# Autodesk Inventor assembly: HopperAssembly_v3
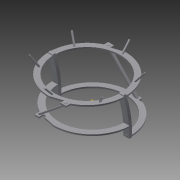
[picture p0: Inventor's stored thumbnail of the model, 180x180]
Saved by Autodesk Inventor 2013 (Build 170138000, 138)
## iProperties
Created: 2013-01-17
Part Number: HopperAssembly_v3
Document SubType Name: Assembly
Designer: twsass
Author: twsass
## Documents named in this file (8)
- E:\Robotics\Hopper\HopperAssembly_v3.iam
- E:\Robotics\Hopper\TopHoopSection_v4.ipt
- E:\Robotics\Hopper\HopperFrontSupport_v2.ipt
- E:\Robotics\Hopper\BottomHoop_v1.ipt
- E:\Robotics\Hopper\MiddleHoop.ipt
- E:\Robotics\Hopper\1Piecelongsupport_v1.ipt
- E:\Robotics\Hopper\1Pieceshortsupport_v1.ipt
- E:\Robotics\Hopper\Funneling_v1.ipt
## Components (14 placed, 7 different names)
1. TopHoopSection_v4:1 — Mate:113, Mate:114, Mate:115, Mate:131, Mate:132, Mate:133, Mate:134, Mate:135, Mate:136, Mate:137, Mate:138, Mate:139
2. HopperFrontSupport_v2:2 — Mate:78, Mate:79, Mate:80, Mate:107, Mate:108, Mate:109, Mate:116, Mate:117, Mate:118
3. TopHoopSection_v4:2 — Mate:116, Mate:117, Mate:118, Mate:122, Mate:123, Mate:124, Mate:125, Mate:126, Mate:127, Mate:128, Mate:129, Mate:130
4. BottomHoop_v1:1 — Mate:64, Mate:65, Mate:66, Mate:78, Mate:79, Mate:80, Mate:87, Mate:119, Mate:120, Mate:121
5. MiddleHoop:1 — Mate:107, Mate:108, Mate:109, Mate:110, Mate:111, Mate:112
6. HopperFrontSupport_v2:3 — Mate:64, Mate:65, Mate:66, Mate:113, Mate:114, Mate:115
7. 1Piecelongsupport_v1:1 — Mate:87, Mate:119, Mate:120, Mate:121
8. 1Pieceshortsupport_v1:1 — Mate:110, Mate:111, Mate:112
9. Funneling_v1:1 — Mate:134, Mate:135, Mate:136
10. Funneling_v1:2 — Mate:122, Mate:123, Mate:124
11. Funneling_v1:3 — Mate:131, Mate:132, Mate:133
12. Funneling_v1:4 — Mate:125, Mate:126, Mate:127
13. Funneling_v1:5 — Mate:137, Mate:138, Mate:139
14. Funneling_v1:6 — Mate:128, Mate:129, Mate:130
## Relationships (40: Mate 40)
- Mate:64: BottomHoop_v1:1 ↔ HopperFrontSupport_v2:3
- Mate:65: BottomHoop_v1:1 ↔ HopperFrontSupport_v2:3
- Mate:66: BottomHoop_v1:1 ↔ HopperFrontSupport_v2:3
- Mate:78: HopperFrontSupport_v2:2 ↔ BottomHoop_v1:1
- Mate:79: HopperFrontSupport_v2:2 ↔ BottomHoop_v1:1
- Mate:80: HopperFrontSupport_v2:2 ↔ BottomHoop_v1:1
- Mate:87: BottomHoop_v1:1 ↔ 1Piecelongsupport_v1:1
- Mate:107: HopperFrontSupport_v2:2 ↔ MiddleHoop:1
- Mate:108: HopperFrontSupport_v2:2 ↔ MiddleHoop:1
- Mate:109: HopperFrontSupport_v2:2 ↔ MiddleHoop:1
- Mate:110: MiddleHoop:1 ↔ 1Pieceshortsupport_v1:1
- Mate:111: MiddleHoop:1 ↔ 1Pieceshortsupport_v1:1
- Mate:112: MiddleHoop:1 ↔ 1Pieceshortsupport_v1:1
- Mate:113: TopHoopSection_v4:1 ↔ HopperFrontSupport_v2:3
- Mate:114: TopHoopSection_v4:1 ↔ HopperFrontSupport_v2:3
- Mate:115: TopHoopSection_v4:1 ↔ HopperFrontSupport_v2:3
- Mate:116: HopperFrontSupport_v2:2 ↔ TopHoopSection_v4:2
- Mate:117: HopperFrontSupport_v2:2 ↔ TopHoopSection_v4:2
- Mate:118: HopperFrontSupport_v2:2 ↔ TopHoopSection_v4:2
- Mate:119: BottomHoop_v1:1 ↔ 1Piecelongsupport_v1:1
- Mate:120: BottomHoop_v1:1 ↔ 1Piecelongsupport_v1:1
- Mate:121: BottomHoop_v1:1 ↔ 1Piecelongsupport_v1:1
- Mate:122: TopHoopSection_v4:2 ↔ Funneling_v1:2
- Mate:123: TopHoopSection_v4:2 ↔ Funneling_v1:2
- Mate:124: TopHoopSection_v4:2 ↔ Funneling_v1:2
- Mate:125: TopHoopSection_v4:2 ↔ Funneling_v1:4
- Mate:126: TopHoopSection_v4:2 ↔ Funneling_v1:4
- Mate:127: TopHoopSection_v4:2 ↔ Funneling_v1:4
- Mate:128: TopHoopSection_v4:2 ↔ Funneling_v1:6
- Mate:129: TopHoopSection_v4:2 ↔ Funneling_v1:6
- Mate:130: TopHoopSection_v4:2 ↔ Funneling_v1:6
- Mate:131: TopHoopSection_v4:1 ↔ Funneling_v1:3
- Mate:132: TopHoopSection_v4:1 ↔ Funneling_v1:3
- Mate:133: TopHoopSection_v4:1 ↔ Funneling_v1:3
- Mate:134: TopHoopSection_v4:1 ↔ Funneling_v1:1
- Mate:135: TopHoopSection_v4:1 ↔ Funneling_v1:1
- Mate:136: TopHoopSection_v4:1 ↔ Funneling_v1:1
- Mate:137: TopHoopSection_v4:1 ↔ Funneling_v1:5
- Mate:138: TopHoopSection_v4:1 ↔ Funneling_v1:5
- Mate:139: TopHoopSection_v4:1 ↔ Funneling_v1:5
